# Autodesk Inventor assembly: SPE31V1 Bisagra
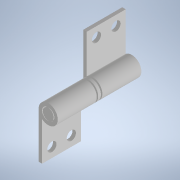
[picture p0: Inventor's stored thumbnail of the model, 180x180]
Saved by Autodesk Inventor 2021.2 (Build 252289000, 289)
## iProperties
Created: 2026-08-14
Part Number: SPE31V1 Bisagra
Document SubType Name: Assembly
Designer: nelso
Author: nelso
## Documents named in this file (4)
- C:\Users\nelso\Desktop\Soporte-Paciente-Espinografia\Workspace\SPE31V1 Bisagra.iam
- C:\Users\nelso\Desktop\Soporte-Paciente-Espinografia\Workspace\SP29V1 Bisagra P1.ipt
- C:\Users\nelso\Desktop\Soporte-Paciente-Espinografia\Workspace\SP30V1 Bisagra P2.ipt
- C:\Users\nelso\Desktop\Soporte-Paciente-Espinografia\Workspace\SP29V1 Bisagra P1_MIR.ipt
## Components (3 placed, 3 different names)
1. SP29V1 Bisagra P1:2 — Mate:2, Mate:4
2. SP30V1 Bisagra P2:1 — Mate:1, Mate:2, Mate:3, Mate:4
3. SP29V1 Bisagra P1_MIR:1 — Mate:1, Mate:3
## Relationships (4: Mate 4)
- Mate:1: SP30V1 Bisagra P2:1 ↔ SP29V1 Bisagra P1_MIR:1
- Mate:2: SP29V1 Bisagra P1:2 ↔ SP30V1 Bisagra P2:1
- Mate:3 (1 mm): SP30V1 Bisagra P2:1 ↔ SP29V1 Bisagra P1_MIR:1
- Mate:4 (1 mm): SP29V1 Bisagra P1:2 ↔ SP30V1 Bisagra P2:1
